# Autodesk Inventor assembly: Assembly1
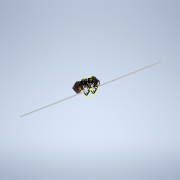
[picture p0: Inventor's stored thumbnail of the model, 180x180]
Saved by Autodesk Inventor 2022 (Build 260153070, 153G)
## iProperties
Created: 2021-07-26
Part Number: Assembly1
Document SubType Name: Assembly
Designer: AKASH ARYAN
Author: AKASH ARYAN
## Documents named in this file (17)
- D:\new\Assembly1.iam
- D:\new\pranshu part.ipt
- D:\new\ashish1.ipt
- D:\new\face.ipt
- D:\new\axel1.ipt
- D:\new\gear holder.ipt
- D:\new\extension circle.ipt
- D:\new\handle.ipt
- D:\new\nut1.ipt
- D:\new\axle small.ipt
- D:\new\gear(1.5 inch with 2mm extra).ipt
- D:\new\bearing.ipt
- D:\new\smalll pin.ipt
- D:\new\boltiii.ipt
- D:\new\dc.ipt
- D:\new\ropeeeeeexxx.ipt
- D:\new\gear(1 inch).ipt
## Components (50 placed, 16 different names)
1. pranshu part:1 — Mate:1, Mate:2, Mate:3, Mate:4, Mate:5, Mate:6, Mate:7, Mate:8, Mate:9, Mate:10, Flush:1, Flush:2, Mate:13, Mate:18, Mate:19, Mate:20, Mate:21, Mate:35, Mate:36, Mate:37, Angle:1, Flush:5, Flush:8, Flush:11, Flush:16, Mate:77, Tangent:8
2. ashish1:1 — Mate:4, Mate:5, Mate:6, Mate:7, Mate:8, Mate:30, Mate:31, Mate:32, Mate:33
3. face:1 — Mate:1, Mate:2, Mate:3
4. axel1:1 — Mate:9, Flush:1, Mate:11, Mate:15, Mate:16, Mate:47, Mate:53, Mate:55, Mate:56, Mate:57
5. axel1:2 — Mate:10, Flush:2, Mate:12, Mate:14, Mate:17, Mate:44, Mate:52, Mate:54, Mate:61, Mate:62
6. gear holder:1 — Mate:11, Mate:12, Mate:13, Mate:34, Mate:38, Mate:39, Mate:40, Mate:41, Mate:42, Mate:43, Flush:3, Flush:4, Mate:48, Mate:50, Mate:51, Flush:6, Flush:7, Flush:9, Flush:10, Flush:12, Flush:13, Flush:14, Flush:15, Mate:76, Mate:78, Flush:17, Mate:81
7. extension circle:1 — Mate:14, Mate:18, Angle:1, Mate:69, Tangent:1, Insert:2
8. extension circle:2 — Mate:15, Mate:19, Mate:24, Mate:27, Mate:68, Tangent:2, Tangent:3
9. extension circle:3 — Mate:16, Mate:20, Mate:23, Mate:28, Mate:66, Tangent:4, Tangent:5
10. extension circle:4 — Mate:17, Mate:21, Mate:67, Tangent:6, Tangent:7, Insert:1
11. handle:1 — Mate:23, Mate:28, Mate:64
12. handle:2 — Insert:2, Mate:75
13. handle:3 — Mate:24, Mate:27, Mate:75
14. handle:4 — Mate:64, Insert:1
15. nut1:1 — Mate:31, Mate:32
16. nut1:2 — Mate:36, Mate:41
17. nut1:3 — Mate:30, Mate:33
18. nut1:6 — Mate:34, Mate:39
19. nut1:7 — Mate:35, Mate:38
20. nut1:9 — Mate:37, Mate:40
21. axle small:1 — Mate:42, Flush:4, Mate:45, Mate:60, Mate:63
22. axle small:2 — Mate:43, Flush:3, Mate:46, Mate:58, Mate:59
23. gear(1.5 inch with 2mm extra):1 — Mate:45, Mate:50
24. gear(1.5 inch with 2mm extra):2 — Mate:46, Mate:48
25. gear(1.5 inch with 2mm extra):3 — Mate:44, Mate:51
26. gear(1.5 inch with 2mm extra):4 — Mate:47, Mate:78
27. bearing:1 — Mate:52, Flush:5
28. bearing:2 — Mate:62, Flush:6
29. bearing:3 — Mate:60, Flush:10
30. bearing:4 — Mate:58, Flush:9
31. bearing:5 — Mate:53, Flush:8
32. bearing:6 — Mate:56, Flush:13
33. bearing:7 — Mate:57, Flush:14
34. bearing:8 — Mate:55, Flush:11
35. bearing:9 — Mate:54, Flush:16
36. bearing:10 — Mate:63, Flush:7
37. bearing:11 — Mate:61, Flush:15
38. bearing:12 — Mate:59, Flush:12
39. smalll pin:1 — Mate:67, Mate:71, Tangent:6
40. smalll pin:2 — Mate:69, Mate:73, Mate:74, Tangent:1
41. smalll pin:3 — Mate:66, Mate:70, Tangent:4
42. smalll pin:4 — Mate:68, Mate:72, Tangent:2
43. boltiii:1 — Mate:73, Mate:74
44. boltiii:2 — Mate:72, Tangent:3
45. boltiii:3 — Mate:70, Tangent:5
46. boltiii:4 — Mate:71, Tangent:7
47. dc:1 — Mate:76, Mate:77, Mate:79, Mate:80
48. bearing:13 — Mate:79, Flush:17
49. ropeeeeeexxx:1 — Tangent:8
50. gear(1 inch):1 — Mate:80, Mate:81
## Relationships (103: Mate 75, Flush 17, Tangent 8, Insert 2, Angle 1)
- Mate:1: pranshu part:1 ↔ face:1
- Mate:2: pranshu part:1 ↔ face:1
- Mate:3: pranshu part:1 ↔ face:1
- Mate:4: pranshu part:1 ↔ ashish1:1
- Mate:5: pranshu part:1 ↔ ashish1:1
- Mate:6: pranshu part:1 ↔ ashish1:1
- Mate:7: pranshu part:1 ↔ ashish1:1
- Mate:8: pranshu part:1 ↔ ashish1:1
- Mate:9: pranshu part:1 ↔ axel1:1
- Mate:10: pranshu part:1 ↔ axel1:2
- Flush:1 (12.7 mm): pranshu part:1 ↔ axel1:1
- Flush:2 (-12.7 mm): pranshu part:1 ↔ axel1:2
- Mate:11: axel1:1 ↔ gear holder:1
- Mate:12: axel1:2 ↔ gear holder:1
- Mate:13 (27.762 mm): pranshu part:1 ↔ gear holder:1
- Mate:14: axel1:2 ↔ extension circle:1
- Mate:15: axel1:1 ↔ extension circle:2
- Mate:16: axel1:1 ↔ extension circle:3
- Mate:17: axel1:2 ↔ extension circle:4
- Mate:18 (1 mm): pranshu part:1 ↔ extension circle:1
- Mate:19 (1 mm): pranshu part:1 ↔ extension circle:2
- Mate:20 (1 mm): pranshu part:1 ↔ extension circle:3
- Mate:21 (1 mm): pranshu part:1 ↔ extension circle:4
- Mate:23: extension circle:3 ↔ handle:1
- Mate:24: extension circle:2 ↔ handle:3
- Mate:27 (1 mm): extension circle:2 ↔ handle:3
- Mate:28 (1 mm): extension circle:3 ↔ handle:1
- Mate:30: ashish1:1 ↔ nut1:3
- Mate:31: ashish1:1 ↔ nut1:1
- Mate:32: ashish1:1 ↔ nut1:1
- Mate:33: ashish1:1 ↔ nut1:3
- Mate:34: gear holder:1 ↔ nut1:6
- Mate:35: pranshu part:1 ↔ nut1:7
- Mate:36: pranshu part:1 ↔ nut1:2
- Mate:37: pranshu part:1 ↔ nut1:9
- Mate:38: gear holder:1 ↔ nut1:7
- Mate:39: gear holder:1 ↔ nut1:6
- Mate:40: gear holder:1 ↔ nut1:9
- Mate:41: gear holder:1 ↔ nut1:2
- Mate:42: gear holder:1 ↔ axle small:1
- Mate:43: gear holder:1 ↔ axle small:2
- Flush:3: gear holder:1 ↔ axle small:2
- Flush:4: gear holder:1 ↔ axle small:1
- Mate:44: axel1:2 ↔ gear(1.5 inch with 2mm extra):3
- Mate:45: axle small:1 ↔ gear(1.5 inch with 2mm extra):1
- Mate:46: axle small:2 ↔ gear(1.5 inch with 2mm extra):2
- Mate:47: axel1:1 ↔ gear(1.5 inch with 2mm extra):4
- Mate:48 (12 mm): gear holder:1 ↔ gear(1.5 inch with 2mm extra):2
- Mate:50 (12 mm): gear holder:1 ↔ gear(1.5 inch with 2mm extra):1
- Mate:51 (12 mm): gear holder:1 ↔ gear(1.5 inch with 2mm extra):3
- Angle:1 (0 deg): pranshu part:1 ↔ extension circle:1
- Mate:52: axel1:2 ↔ bearing:1
- Mate:53: axel1:1 ↔ bearing:5
- Mate:54: axel1:2 ↔ bearing:9
- Mate:55: axel1:1 ↔ bearing:8
- Mate:56: axel1:1 ↔ bearing:6
- Mate:57: axel1:1 ↔ bearing:7
- Mate:58: axle small:2 ↔ bearing:4
- Mate:59: axle small:2 ↔ bearing:12
- Mate:60: axle small:1 ↔ bearing:3
- Mate:61: axel1:2 ↔ bearing:11
- Mate:62: axel1:2 ↔ bearing:2
- Mate:63: axle small:1 ↔ bearing:10
- Flush:5 (1 mm): pranshu part:1 ↔ bearing:1
- Flush:6 (1 mm): gear holder:1 ↔ bearing:2
- Flush:7 (1 mm): gear holder:1 ↔ bearing:10
- Flush:8 (1 mm): pranshu part:1 ↔ bearing:5
- Flush:9 (1 mm): gear holder:1 ↔ bearing:4
- Flush:10 (1 mm): gear holder:1 ↔ bearing:3
- Flush:11 (1 mm): pranshu part:1 ↔ bearing:8
- Flush:12 (1 mm): gear holder:1 ↔ bearing:12
- Flush:13 (1 mm): gear holder:1 ↔ bearing:6
- Flush:14 (1 mm): gear holder:1 ↔ bearing:7
- Flush:15 (-1 mm): gear holder:1 ↔ bearing:11
- Mate:64 (120 mm): handle:1 ↔ handle:4
- Mate:66: extension circle:3 ↔ smalll pin:3
- Mate:67: extension circle:4 ↔ smalll pin:1
- Mate:68: extension circle:2 ↔ smalll pin:4
- Mate:69: extension circle:1 ↔ smalll pin:2
- Flush:16 (-1 mm): pranshu part:1 ↔ bearing:9
- Mate:70: smalll pin:3 ↔ boltiii:3
- Mate:71: smalll pin:1 ↔ boltiii:4
- Mate:72: smalll pin:4 ↔ boltiii:2
- Mate:73: smalll pin:2 ↔ boltiii:1
- Mate:74 (3.7 mm): smalll pin:2 ↔ boltiii:1
- Tangent:1: extension circle:1 ↔ smalll pin:2
- Tangent:2: extension circle:2 ↔ smalll pin:4
- Tangent:3: extension circle:2 ↔ boltiii:2
- Tangent:4: extension circle:3 ↔ smalll pin:3
- Tangent:5: extension circle:3 ↔ boltiii:3
- Tangent:6: extension circle:4 ↔ smalll pin:1
- Tangent:7: extension circle:4 ↔ boltiii:4
- Insert:1 (8 mm): extension circle:4 ↔ handle:4
- Insert:2 (8 mm): extension circle:1 ↔ handle:2
- Mate:75 (120 mm): handle:2 ↔ handle:3
- Mate:76: gear holder:1 ↔ dc:1
- Mate:77 (4 mm): pranshu part:1 ↔ dc:1
- Mate:78 (12 mm): gear holder:1 ↔ gear(1.5 inch with 2mm extra):4
- Mate:79: dc:1 ↔ bearing:13
- Flush:17 (-1 mm): gear holder:1 ↔ bearing:13
- Tangent:8 (150 mm): pranshu part:1 ↔ ropeeeeeexxx:1
- Mate:80: dc:1 ↔ gear(1 inch):1
- Mate:81 (12 mm): gear holder:1 ↔ gear(1 inch):1
